# Autodesk Inventor assembly: alternativeJoint_ams
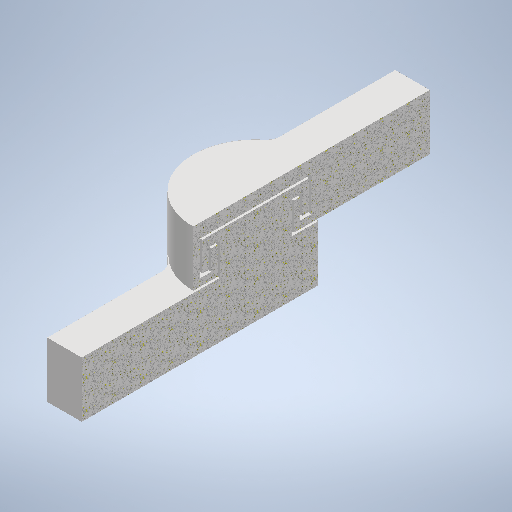
[picture p0: Inventor's stored thumbnail of the model, 512x512]
Saved by Autodesk Inventor 2025.1 (Build 291241000, 241)
## iProperties
Created: 2024-11-07
Part Number: alternativeJoint_ams
Document SubType Name: Assembly
Designer: ZOMBULLI
Author: ZOMBULLI
## Documents named in this file (3)
- C:\Users\zombulli\OneDrive - Carl Zeiss AG\Desktop\DHBW\Semester 5\mte380\Stewart Platform_new\alternativeJoint_ams.iam
- C:\Users\zombulli\OneDrive - Carl Zeiss AG\Desktop\DHBW\Semester 5\mte380\Stewart Platform_new\print testing\alternativeJoint.ipt
- C:\Users\zombulli\OneDrive - Carl Zeiss AG\Desktop\DHBW\Semester 5\mte380\Stewart Platform_new\print testing\alternativeJoint2.ipt
## Components (2 placed, 2 different names)
1. alternativeJoint:1 — Passend:1, Passend:2, Passend:3
2. alternativeJoint2:1 — Passend:1, Passend:2, Passend:3
## Relationships (3: Mate 3)
- Passend:1 [Mate] (0.3 mm): alternativeJoint:1 ↔ alternativeJoint2:1
- Passend:2 [Mate]: alternativeJoint:1 ↔ alternativeJoint2:1
- Passend:3 [Mate]: alternativeJoint:1 ↔ alternativeJoint2:1
